# Autodesk Inventor assembly: Bevel_Ass
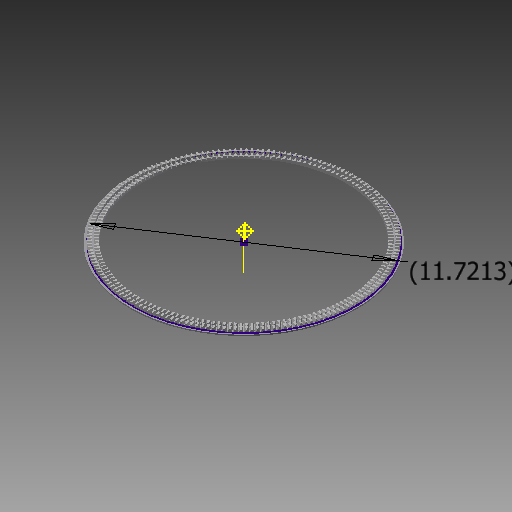
[picture p0: Inventor's stored thumbnail of the model, 512x512]
Saved by Autodesk Inventor 2017 (Build 210142000, 142)
## iProperties
Created: 2017-01-26
Part Number: Bevel_Ass
Document SubType Name: Assembly
Designer: David Kopala
Author: David Kopala
## Documents named in this file (4)
- Z:\Documents\Drone\Drone\3D Models\Project\Chassis_04\Bevel_Ass.iam
- Z:\Documents\Drone\Drone\3D Models\Project\Chassis_04\BevelBasePlate.ipt
- Z:\Documents\Drone\Drone\3D Models\Project\Chassis_04\BevelGear_Ref\Design Accelerator\Bevel Gear13.ipt
- Z:\Documents\Drone\Drone\3D Models\Project\Chassis_04\BevelOuter_Ref\Design Accelerator\Bevel Gear11.ipt
## Components (3 placed, 2 different names)
1. BevelBasePlate:1 — Insert:1
2. Bevel Gear1:1 — Insert:1, Insert:2
3. Bevel Gear1:2 — Insert:2
## Relationships (2: Insert 2)
- Insert:1: BevelBasePlate:1 ↔ Bevel Gear1:1
- Insert:2: Bevel Gear1:1 ↔ Bevel Gear1:2
